# Autodesk Inventor assembly: full
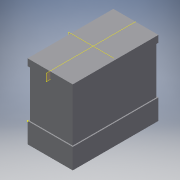
[picture p0: Inventor's stored thumbnail of the model, 180x180]
Saved by Autodesk Inventor 2017 (Build 210142000, 142)
## iProperties
Created: 2019-05-03
Part Number: full
Document SubType Name: Assembly
Designer: Roman
Author: Roman
## Documents named in this file (5)
- C:\Users\Roman\Documents\CAD\enclosure rev1\full.iam
- C:\Users\Roman\Documents\CAD\enclosure rev1\rev1 base.ipt
- C:\Users\Roman\Documents\CAD\enclosure rev1\rev1 small wall.ipt
- C:\Users\Roman\Documents\CAD\enclosure rev1\rev1 large wall.ipt
- C:\Users\Roman\Documents\CAD\enclosure rev1\rev1 top.ipt
## Components (6 placed, 4 different names)
1. rev1 base:1 — Mate:1, Mate:2, Mate:3, Mate:4, Mate:5, Mate:6, Mate:7, Mate:8, Mate:9, Mate:10, Mate:11, Mate:12
2. rev1 large wall:1 — Mate:4, Mate:5, Mate:6, Mate:15
3. rev1 large wall:2 — Mate:1, Mate:2, Mate:3
4. rev1 small wall:1 — Mate:10, Mate:11, Mate:12, Mate:13, Mate:14
5. rev1 small wall:2 — Mate:7, Mate:8, Mate:9
6. rev1 top:1 — Mate:13, Mate:14, Mate:15
## Relationships (15: Mate 15)
- Mate:1: rev1 base:1 ↔ rev1 large wall:2
- Mate:2: rev1 base:1 ↔ rev1 large wall:2
- Mate:3: rev1 base:1 ↔ rev1 large wall:2
- Mate:4: rev1 base:1 ↔ rev1 large wall:1
- Mate:5: rev1 base:1 ↔ rev1 large wall:1
- Mate:6: rev1 base:1 ↔ rev1 large wall:1
- Mate:7: rev1 base:1 ↔ rev1 small wall:2
- Mate:8: rev1 base:1 ↔ rev1 small wall:2
- Mate:9: rev1 base:1 ↔ rev1 small wall:2
- Mate:10: rev1 base:1 ↔ rev1 small wall:1
- Mate:11: rev1 base:1 ↔ rev1 small wall:1
- Mate:12: rev1 base:1 ↔ rev1 small wall:1
- Mate:13: rev1 small wall:1 ↔ rev1 top:1
- Mate:14: rev1 small wall:1 ↔ rev1 top:1
- Mate:15: rev1 large wall:1 ↔ rev1 top:1
